# Autodesk Inventor assembly: Assembly
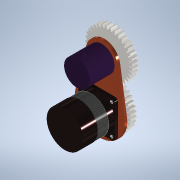
[picture p0: Inventor's stored thumbnail of the model, 180x180]
Saved by Autodesk Inventor 2020 (Build 240168000, 168)
## iProperties
Created: 2021-06-11
Part Number: Assembly
Document SubType Name: Assembly
Designer: user
Author: user
## Documents named in this file (5)
- C:\Users\user\Documents\GitHub\adaptive_contrrol\adaptive_control\odrive\CAD\Assembly.iam
- C:\Users\user\Documents\GitHub\adaptive_contrrol\adaptive_control\odrive\CAD\57type_BLDC_motor\BLDC_motor.ipt
- C:\Users\user\Documents\GitHub\adaptive_contrrol\adaptive_control\odrive\CAD\Encoder\E6B2-CWZ6C.ipt
- C:\Users\user\Documents\GitHub\adaptive_contrrol\adaptive_control\odrive\CAD\Encoder\Linker_Structure.ipt
- C:\Users\user\Documents\GitHub\adaptive_contrrol\adaptive_control\odrive\CAD\Assembly\機械便覽魔法師\正齒輪1.iam
## Components (4 placed, 4 different names)
1. BLDC_motor:1 — 齊平:1, 貼合:1, 貼合:2, 貼合:3
2. E6B2-CWZ6C:1 — 齊平:1, 齊平:2, 貼合:1, 貼合:4
3. Linker_Structure:1 — 齊平:2, 貼合:5
4. 正齒輪:1 [sub-assembly] — 貼合:2, 貼合:3, 貼合:4, 貼合:5
## Relationships (7: Mate 5, Flush 2)
- 齊平:1 [Flush]: BLDC_motor:1 ↔ E6B2-CWZ6C:1
- 齊平:2 [Flush]: E6B2-CWZ6C:1 ↔ Linker_Structure:1
- 貼合:1 [Mate] (70 mm): BLDC_motor:1 ↔ E6B2-CWZ6C:1
- 貼合:2 [Mate]: BLDC_motor:1 ↔ 正齒輪:1
- 貼合:3 [Mate] (10 mm): BLDC_motor:1 ↔ 正齒輪:1
- 貼合:4 [Mate]: E6B2-CWZ6C:1 ↔ 正齒輪:1
- 貼合:5 [Mate] (7 mm): Linker_Structure:1 ↔ 正齒輪:1
